# Autodesk Inventor assembly: plytka_dol
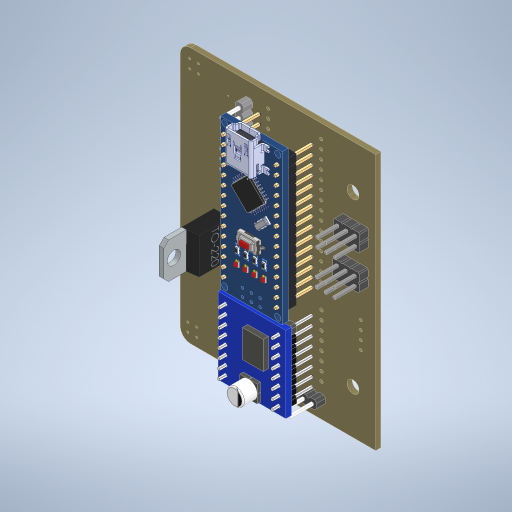
[picture p0: Inventor's stored thumbnail of the model, 512x512]
Saved by Autodesk Inventor 2023 (Build 270158000, 158)
## iProperties
Created: 2023-07-07
Part Number: plytka_dol
Document SubType Name: Assembly
Designer: Kamil
Author: Kamil
## Documents named in this file (8)
- C:\Users\Kamil\Desktop\MojeRoboty\Stefan\mechanics 2\plytka_dol.iam
- C:\Users\Kamil\Desktop\MojeRoboty\Stefan\mechanics 2\Board_1.ipt
- C:\Users\Kamil\Desktop\MojeRoboty\Stefan\mechanics 2\motor drive module TB6612.ipt
- C:\Users\Kamil\Desktop\MojeRoboty\Stefan\mechanics 2\ARDUINO_NANO.ipt
- C:\Users\Kamil\Desktop\MojeRoboty\Stefan\mechanics 2\1X02.ipt
- C:\Users\Kamil\Desktop\MojeRoboty\Stefan\mechanics 2\1X03.ipt
- C:\Users\Kamil\Desktop\MojeRoboty\Stefan\mechanics 2\2X03.ipt
- C:\Users\Kamil\Desktop\MojeRoboty\Stefan\mechanics 2\TO220V.ipt
## Components (10 placed, 7 different names)
1. Board_1:1 — Zestawiające:1, Równoległe:1, Równoległe:2, Zestawiające:2, Zestawiające:3, Zestawiające:4, Zestawiające:5, Zestawiające:6, Zestawiające:7, Zestawiające:8, Zestawiające:9
2. motor drive module TB6612:1 — Zestawiające:2
3. ARDUINO_NANO:1 — Zestawiające:1, Równoległe:1, Równoległe:2
4. 1X02:1 — Zestawiające:6
5. 1X03:1 — Zestawiające:9
6. 2X03:1 — Zestawiające:5
7. TO220V:1 — Zestawiające:3
8. 2X03:2 — Zestawiające:4
9. 1X02:2 — Zestawiające:7
10. 1X03:2 — Zestawiające:8
## Relationships (11: Mate 9, Flush 2)
- Zestawiające:1 [Mate] (8.4 mm): Board_1:1 ↔ ARDUINO_NANO:1
- Równoległe:1 [Flush] (-0.22 mm): Board_1:1 ↔ ARDUINO_NANO:1
- Równoległe:2 [Flush] (14.408 mm): Board_1:1 ↔ ARDUINO_NANO:1
- Zestawiające:2 [Mate] (8.4 mm): Board_1:1 ↔ motor drive module TB6612:1
- Zestawiające:3 [Mate] (5 mm): Board_1:1 ↔ TO220V:1
- Zestawiające:4 [Mate]: Board_1:1 ↔ 2X03:2
- Zestawiające:5 [Mate]: Board_1:1 ↔ 2X03:1
- Zestawiające:6 [Mate]: Board_1:1 ↔ 1X02:1
- Zestawiające:7 [Mate]: Board_1:1 ↔ 1X02:2
- Zestawiające:8 [Mate]: Board_1:1 ↔ 1X03:2
- Zestawiające:9 [Mate]: Board_1:1 ↔ 1X03:1
